# Autodesk Inventor assembly: Final_Assembly
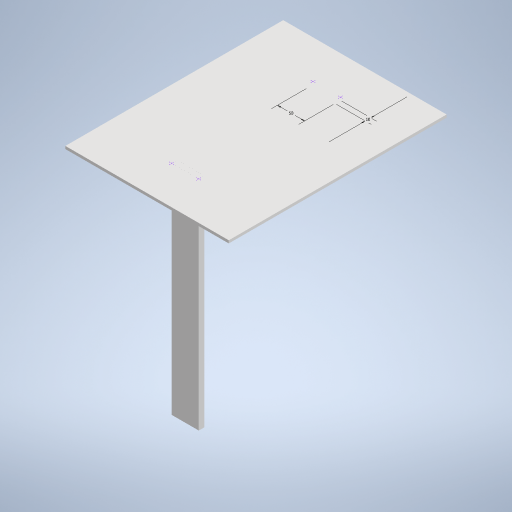
[picture p0: Inventor's stored thumbnail of the model, 512x512]
Saved by Autodesk Inventor 2024 (Build 280153000, 153)
## iProperties
Created: 2023-08-27
Part Number: Final_Assembly
Document SubType Name: Assembly
Designer: katch
Author: katch
## Documents named in this file (3)
- C:\Users\91865\Downloads\Final_Assembly.iam
- C:\Users\91865\Downloads\BasePlate.ipt
- C:\Users\91865\Downloads\pillar.ipt
## Components (2 placed, 2 different names)
1. BasePlate:1 — Rigid:1
2. pillar:1 — Rigid:1
## Relationships (1: WeldJoint 1)
- Rigid:1 [WeldJoint]: BasePlate:1 ↔ pillar:1
